# Autodesk Inventor assembly: WinderAssembly
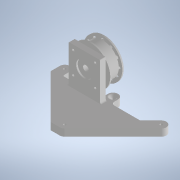
[picture p0: Inventor's stored thumbnail of the model, 180x180]
Saved by Autodesk Inventor 2020.2 (Build 242310000, 310)
## iProperties
Created: 2020-03-15
Part Number: WinderAssembly
Document SubType Name: Assembly
Designer: elmar
Author: elmar
## Documents named in this file (3)
- C:\Users\elmar\OneDrive\Inventor\FourWireBraidingMachine\WinderAssembly.iam
- C:\Users\elmar\OneDrive\Inventor\FourWireBraidingMachine\WinderSpool.ipt
- C:\Users\elmar\OneDrive\Inventor\FourWireBraidingMachine\FourWireWinderBracket.ipt
## Components (2 placed, 2 different names)
1. WinderSpool:1 — Insert:1
2. FourWireWinderBracket:1 — Insert:1
## Relationships (1: Insert 1)
- Insert:1 (1 mm): WinderSpool:1 ↔ FourWireWinderBracket:1
